# Autodesk Inventor assembly: Сборка1+-
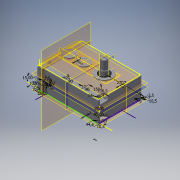
[picture p0: Inventor's stored thumbnail of the model, 180x180]
Saved by Autodesk Inventor 2018 (Build 220112000, 112)
## iProperties
Created: 2018-03-25
Part Number: Сборка1+-
Material: Типовые
Document SubType Name: Assembly
Designer: kriku
Mass: 8188.81 g
Surface Area: 16132 cm^2
Volume: 6448.11 cm^3
Density: 1.26995 g/cm^3
Author: kriku
## Documents named in this file (22)
- C:\Users\kriku\OneDrive\Рабочий стол\6 семестр\курсач ДМ\deadmash\Куча инви\Сборка1+-.iam
- C:\Users\kriku\OneDrive\Рабочий стол\6 семестр\курсач ДМ\deadmash\Куча инви\Вал быстроходный.ipt
- C:\Users\kriku\OneDrive\Рабочий стол\6 семестр\курсач ДМ\deadmash\Куча инви\Колесо быстроходное.ipt
- C:\Users\kriku\OneDrive\Рабочий стол\6 семестр\курсач ДМ\deadmash\Куча инви\Вал переходный.ipt
- C:\Users\kriku\OneDrive\Рабочий стол\6 семестр\курсач ДМ\deadmash\Куча инви\Колесл тихоходное.ipt
- C:\Users\kriku\OneDrive\Рабочий стол\6 семестр\курсач ДМ\deadmash\Куча инви\Вал тихоходный.ipt
- C:\Users\kriku\OneDrive\Документы\Inventor\Content Center Files\R2018\ru-RU\GOST 8338-75\Подшипник 206 ГОСТ 8338-75.ipt
- C:\Users\kriku\OneDrive\Документы\Inventor\Content Center Files\R2018\ru-RU\GOST 8338-75\Подшипник 211 ГОСТ 8338-75.ipt
- C:\Users\kriku\OneDrive\Рабочий стол\6 семестр\курсач ДМ\deadmash\Куча инви\Сборка1\Мастер проектирования\Шпоночное соединение1.iam
- C:\Users\kriku\OneDrive\Рабочий стол\6 семестр\курсач ДМ\Куча инви\Крышка обычная на 30.ipt
- C:\Users\kriku\OneDrive\Рабочий стол\6 семестр\курсач ДМ\Куча инви\Крышка обычная на 55.ipt
- C:\Users\kriku\OneDrive\Рабочий стол\6 семестр\курсач ДМ\Куча инви\Крышка сквозная на 55.ipt
- C:\Users\kriku\OneDrive\Документы\Inventor\Content Center Files\R2018\ru-RU\GOST 8752-79(1)\Манжет 1-55x80x8 ГОСТ 8752-79.ipt
- C:\Users\kriku\OneDrive\Рабочий стол\6 семестр\курсач ДМ\Куча инви\Крышка сквозная на 30.ipt
- C:\Users\kriku\OneDrive\Документы\Inventor\Content Center Files\R2018\ru-RU\GOST 8752-79(1)\Манжет 1-30x47x7 ГОСТ 8752-79.ipt
- C:\Users\kriku\OneDrive\Рабочий стол\6 семестр\курсач ДМ\Куча инви\заплечик быстроход меньший.ipt
- C:\Users\kriku\OneDrive\Рабочий стол\6 семестр\курсач ДМ\Куча инви\заплечик переходный.ipt
- C:\Users\kriku\OneDrive\Рабочий стол\6 семестр\курсач ДМ\Куча инви\заплечик переходный  кряком.ipt
- C:\Users\kriku\OneDrive\Рабочий стол\6 семестр\курсач ДМ\Куча инви\плюс к быстроходному.ipt
- C:\Users\kriku\OneDrive\Рабочий стол\6 семестр\курсач ДМ\deadmash\Куча инви\между крышкой и подшипником.ipt
- C:\Users\kriku\OneDrive\Рабочий стол\6 семестр\курсач ДМ\Куча инви\Корпус.ipt
- C:\Users\kriku\OneDrive\Рабочий стол\6 семестр\курсач ДМ\deadmash\Куча инви\gost\Винт M6-6gx16 ГОСТ 11738-84.ipt
## Components (30 placed, 21 different names)
1. Вал быстроходный:1 — Совмещение:1, Совмещение:2, Совмещение:11, Совмещение:17, Заподлицо:7, Заподлицо:8, Заподлицо:10, Совмещение:36, Жесткий:1, Совмещение:67
2. Колесо быстроходное:1 — Заподлицо:1, Совмещение:1, Совмещение:2, Совмещение:3, Совмещение:4, Совмещение:5, Угол:2, С поворотом:5
3. Вал переходный:1 — Совмещение:3, Совмещение:4, Совмещение:5, Совмещение:6, Совмещение:7, Совмещение:8, Совмещение:13, Совмещение:14, Совмещение:18, Совмещение:23, Заподлицо:3, Угол:1, Совмещение:24, Угол:2, Заподлицо:4, Заподлицо:5, Совмещение:26, Заподлицо:6, Совмещение:32, Совмещение:33, Вставка:1, Совмещение:50, Цилиндрический:2, Совмещение:63
4. Колесл тихоходное:1 — Совмещение:6, Совмещение:7, Совмещение:8, Заподлицо:2, Совмещение:32, Совмещение:33, Заподлицо:20, Совмещение:49, Совмещение:50, Совмещение:51, Совмещение:57
5. Вал тихоходный:1 — Заподлицо:2, Совмещение:29, Совмещение:30, Совмещение:34, Заподлицо:9, Заподлицо:20, Совмещение:49, Совмещение:51, Совмещение:52, Совмещение:59
6. Подшипник ГОСТ 8338-75 206:1 — Совмещение:11, Совмещение:17, Совмещение:28, Совмещение:42, Совмещение:62
7. Подшипник ГОСТ 8338-75 206:2 — Совмещение:48, Совмещение:67
8. Подшипник ГОСТ 8338-75 206:3 — Совмещение:13, Совмещение:18, Совмещение:25, Совмещение:40, Совмещение:61
9. Подшипник ГОСТ 8338-75 206:4 — Совмещение:14, Совмещение:23, Совмещение:27, Совмещение:45, Цилиндрический:2, С поворотом:7
10. Шпоночное соединение:1 [sub-assembly] — Заподлицо:3, Угол:1, Совмещение:24
11. Крышка обычная на 30:1 — Заподлицо:4, Заподлицо:5, Совмещение:25, Заподлицо:12, Заподлицо:13, Совмещение:39, Совмещение:66, Допуск симметричности:1
12. Крышка обычная на 30:2 — Совмещение:26, Заподлицо:6, Совмещение:27, Заподлицо:16, Совмещение:43, Совмещение:44, Допуск симметричности:1
13. Крышка обычная на 30:3 — Заподлицо:7, Заподлицо:8, Совмещение:28, Заподлицо:14, Заподлицо:15, Совмещение:41
14. Крышка обычная на 55:1 — Совмещение:29, Совмещение:30, Совмещение:56, Совмещение:69
15. Крышка сквозная на 55:1 — Совмещение:34, Заподлицо:9, Заподлицо:17, Заподлицо:21, Совмещение:68
16. Манжет 1 ГОСТ 8752-79 55 x 80 x 8:1 — Заподлицо:17, Заподлицо:21
17. Крышка сквозная на 30:1 — С поворотом:2, Заподлицо:10, Совмещение:36, Заподлицо:18, Заподлицо:19, Совмещение:46, Совмещение:47
18. Манжет 1 ГОСТ 8752-79 30 x 47 x 7:1 — С поворотом:2, Заподлицо:18
19. заплечик быстроход меньший:1 — С поворотом:6, Совмещение:57
20. заплечик переходный:1 — С поворотом:5, Совмещение:61
21. заплечик переходный  кряком:1 — Вставка:1, С поворотом:7, Совмещение:63
22. плюс к быстроходному:1 — Жесткий:1, Совмещение:62
23. между крышкой и подшипником:1 — Заподлицо:12, Заподлицо:13, Совмещение:39, Совмещение:40
24. между крышкой и подшипником:2 — Заподлицо:14, Заподлицо:15, Совмещение:41, Совмещение:42
25. между крышкой и подшипником:3 — Заподлицо:16, Совмещение:43, Совмещение:44, Совмещение:45
26. между крышкой и подшипником:4 — Заподлицо:19, Совмещение:46, Совмещение:47, Совмещение:48
27. Подшипник ГОСТ 8338-75 211:1 — Совмещение:52, С поворотом:6, Совмещение:56
28. Подшипник ГОСТ 8338-75 211:2 — Совмещение:59, Цилиндрический:3, Совмещение:68
29. Корпус:1 — Совмещение:66, Заподлицо:22, Цилиндрический:3, Совмещение:69
30. Винт M6-6gx16 ГОСТ 11738-84:1
## Relationships (82: Mate 49, Flush 22, RevoluteJoint 4, Angle 2, CylindricalJoint 2, Insert 1, WeldJoint 1, Symmetry 1)
- Заподлицо:1 [Flush]: Колесо быстроходное:1
- Совмещение:1 [Mate] (110 mm): Вал быстроходный:1 ↔ Колесо быстроходное:1
- Совмещение:2 [Mate]: Вал быстроходный:1 ↔ Колесо быстроходное:1
- Совмещение:3 [Mate]: Колесо быстроходное:1 ↔ Вал переходный:1
- Совмещение:4 [Mate]: Колесо быстроходное:1 ↔ Вал переходный:1
- Совмещение:5 [Mate]: Колесо быстроходное:1 ↔ Вал переходный:1
- Совмещение:6 [Mate]: Вал переходный:1 ↔ Колесл тихоходное:1
- Совмещение:7 [Mate]: Вал переходный:1 ↔ Колесл тихоходное:1
- Совмещение:8 [Mate] (150 mm): Вал переходный:1 ↔ Колесл тихоходное:1
- Заподлицо:2 [Flush]: Колесл тихоходное:1 ↔ Вал тихоходный:1
- Совмещение:11 [Mate]: Вал быстроходный:1 ↔ Подшипник ГОСТ 8338-75 206:1
- Совмещение:13 [Mate]: Вал переходный:1 ↔ Подшипник ГОСТ 8338-75 206:3
- Совмещение:14 [Mate]: Вал переходный:1 ↔ Подшипник ГОСТ 8338-75 206:4
- Совмещение:17 [Mate]: Вал быстроходный:1 ↔ Подшипник ГОСТ 8338-75 206:1
- Совмещение:18 [Mate]: Вал переходный:1 ↔ Подшипник ГОСТ 8338-75 206:3
- Совмещение:23 [Mate]: Вал переходный:1 ↔ Подшипник ГОСТ 8338-75 206:4
- Заподлицо:3 [Flush] (16 mm): Вал переходный:1 ↔ Шпоночное соединение:1
- Угол:1 [Angle] (180 deg): Вал переходный:1 ↔ Шпоночное соединение:1
- Совмещение:24 [Mate]: Вал переходный:1 ↔ Шпоночное соединение:1
- Угол:2 [Angle] (90 deg): Колесо быстроходное:1 ↔ Вал переходный:1
- Заподлицо:4 [Flush]: Вал переходный:1 ↔ Крышка обычная на 30:1
- Заподлицо:5 [Flush]: Вал переходный:1 ↔ Крышка обычная на 30:1
- Совмещение:25 [Mate]: Подшипник ГОСТ 8338-75 206:3 ↔ Крышка обычная на 30:1
- Совмещение:26 [Mate]: Вал переходный:1 ↔ Крышка обычная на 30:2
- Заподлицо:6 [Flush]: Вал переходный:1 ↔ Крышка обычная на 30:2
- Совмещение:27 [Mate]: Подшипник ГОСТ 8338-75 206:4 ↔ Крышка обычная на 30:2
- Заподлицо:7 [Flush]: Вал быстроходный:1 ↔ Крышка обычная на 30:3
- Заподлицо:8 [Flush]: Вал быстроходный:1 ↔ Крышка обычная на 30:3
- Совмещение:28 [Mate]: Подшипник ГОСТ 8338-75 206:1 ↔ Крышка обычная на 30:3
- Совмещение:29 [Mate]: Вал тихоходный:1 ↔ Крышка обычная на 55:1
- Совмещение:30 [Mate]: Вал тихоходный:1 ↔ Крышка обычная на 55:1
- Совмещение:32 [Mate]: Вал переходный:1 ↔ Колесл тихоходное:1
- Совмещение:33 [Mate]: Вал переходный:1 ↔ Колесл тихоходное:1
- Совмещение:34 [Mate]: Вал тихоходный:1 ↔ Крышка сквозная на 55:1
- Заподлицо:9 [Flush]: Вал тихоходный:1 ↔ Крышка сквозная на 55:1
- С поворотом:2 [RevoluteJoint]: Крышка сквозная на 30:1 ↔ Манжет 1 ГОСТ 8752-79 30 x 47 x 7:1
- Заподлицо:10 [Flush]: Вал быстроходный:1 ↔ Крышка сквозная на 30:1
- Совмещение:36 [Mate]: Вал быстроходный:1 ↔ Крышка сквозная на 30:1
- С поворотом:5 [RevoluteJoint]: Колесо быстроходное:1 ↔ заплечик переходный:1
- Вставка:1 [Insert]: Вал переходный:1 ↔ заплечик переходный  кряком:1
- Жесткий:1 [WeldJoint]: Вал быстроходный:1 ↔ плюс к быстроходному:1
- Заподлицо:11 [Flush] (60 mm)
- Заподлицо:12 [Flush]: Крышка обычная на 30:1 ↔ между крышкой и подшипником:1
- Заподлицо:13 [Flush]: Крышка обычная на 30:1 ↔ между крышкой и подшипником:1
- Совмещение:39 [Mate]: Крышка обычная на 30:1 ↔ между крышкой и подшипником:1
- Совмещение:40 [Mate]: Подшипник ГОСТ 8338-75 206:3 ↔ между крышкой и подшипником:1
- Заподлицо:14 [Flush]: Крышка обычная на 30:3 ↔ между крышкой и подшипником:2
- Заподлицо:15 [Flush]: Крышка обычная на 30:3 ↔ между крышкой и подшипником:2
- Совмещение:41 [Mate]: Крышка обычная на 30:3 ↔ между крышкой и подшипником:2
- Совмещение:42 [Mate]: Подшипник ГОСТ 8338-75 206:1 ↔ между крышкой и подшипником:2
- Заподлицо:16 [Flush]: Крышка обычная на 30:2 ↔ между крышкой и подшипником:3
- Совмещение:43 [Mate]: Крышка обычная на 30:2 ↔ между крышкой и подшипником:3
- Совмещение:44 [Mate]: Крышка обычная на 30:2 ↔ между крышкой и подшипником:3
- Совмещение:45 [Mate]: Подшипник ГОСТ 8338-75 206:4 ↔ между крышкой и подшипником:3
- Заподлицо:17 [Flush]: Крышка сквозная на 55:1 ↔ Манжет 1 ГОСТ 8752-79 55 x 80 x 8:1
- Заподлицо:18 [Flush]: Крышка сквозная на 30:1 ↔ Манжет 1 ГОСТ 8752-79 30 x 47 x 7:1
- Заподлицо:19 [Flush]: Крышка сквозная на 30:1 ↔ между крышкой и подшипником:4
- Совмещение:46 [Mate]: Крышка сквозная на 30:1 ↔ между крышкой и подшипником:4
- Совмещение:47 [Mate]: Крышка сквозная на 30:1 ↔ между крышкой и подшипником:4
- Совмещение:48 [Mate]: Подшипник ГОСТ 8338-75 206:2 ↔ между крышкой и подшипником:4
- Заподлицо:20 [Flush]: Колесл тихоходное:1 ↔ Вал тихоходный:1
- Совмещение:49 [Mate]: Колесл тихоходное:1 ↔ Вал тихоходный:1
- Совмещение:50 [Mate]: Вал переходный:1 ↔ Колесл тихоходное:1
- Совмещение:51 [Mate]: Колесл тихоходное:1 ↔ Вал тихоходный:1
- Совмещение:52 [Mate]: Вал тихоходный:1 ↔ Подшипник ГОСТ 8338-75 211:1
- С поворотом:6 [RevoluteJoint]: заплечик быстроход меньший:1 ↔ Подшипник ГОСТ 8338-75 211:1
- Совмещение:56 [Mate]: Крышка обычная на 55:1 ↔ Подшипник ГОСТ 8338-75 211:1
- Совмещение:57 [Mate]: Колесл тихоходное:1 ↔ заплечик быстроход меньший:1
- Заподлицо:21 [Flush]: Крышка сквозная на 55:1 ↔ Манжет 1 ГОСТ 8752-79 55 x 80 x 8:1
- Совмещение:59 [Mate]: Вал тихоходный:1 ↔ Подшипник ГОСТ 8338-75 211:2
- Совмещение:61 [Mate]: Подшипник ГОСТ 8338-75 206:3 ↔ заплечик переходный:1
- Совмещение:62 [Mate]: Подшипник ГОСТ 8338-75 206:1 ↔ плюс к быстроходному:1
- Цилиндрический:2 [CylindricalJoint]: Вал переходный:1 ↔ Подшипник ГОСТ 8338-75 206:4
- С поворотом:7 [RevoluteJoint]: Подшипник ГОСТ 8338-75 206:4 ↔ заплечик переходный  кряком:1
- Совмещение:63 [Mate]: Вал переходный:1 ↔ заплечик переходный  кряком:1
- Совмещение:66 [Mate]: Крышка обычная на 30:1 ↔ Корпус:1
- Совмещение:67 [Mate]: Вал быстроходный:1 ↔ Подшипник ГОСТ 8338-75 206:2
- Заподлицо:22 [Flush]: Корпус:1
- Цилиндрический:3 [CylindricalJoint]: Подшипник ГОСТ 8338-75 211:2 ↔ Корпус:1
- Совмещение:68 [Mate]: Крышка сквозная на 55:1 ↔ Подшипник ГОСТ 8338-75 211:2
- Допуск симметричности:1 [Symmetry]: Крышка обычная на 30:1 ↔ Крышка обычная на 30:2
- Совмещение:69 [Mate]: Крышка обычная на 55:1 ↔ Корпус:1
